# Autodesk Inventor assembly: Ensamblaje
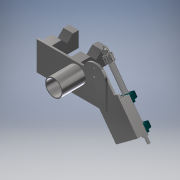
[picture p0: Inventor's stored thumbnail of the model, 180x180]
Saved by Autodesk Inventor 2018 (Build 220112000, 112)
## iProperties
Created: 2021-07-05
Part Number: Ensamblaje
Material: Genérico
Document SubType Name: Assembly
Designer: GABRIEL
Author: GABRIEL
## Documents named in this file (9)
- C:\Users\GABRIEL\Documents\Gabriel\UNAL\SEMESTRE XI\Automatización de PM\Proyecto\Maquina de boca de pescado\Ensamblaje.iam
- C:\Users\GABRIEL\Documents\Gabriel\Modelados\Placa1.ipt
- C:\Users\GABRIEL\Documents\Gabriel\UNAL\SEMESTRE XI\Automatización de PM\Proyecto\Maquina de boca de pescado\Base.ipt
- C:\Users\GABRIEL\Documents\Gabriel\UNAL\SEMESTRE XI\Automatización de PM\Proyecto\Maquina de boca de pescado\Posicionador.ipt
- C:\Users\GABRIEL\Documents\Gabriel\UNAL\SEMESTRE XI\Automatización de PM\Proyecto\Maquina de boca de pescado\pie.ipt
- C:\Users\GABRIEL\Documents\Gabriel\UNAL\SEMESTRE XI\Automatización de PM\Proyecto\Maquina de boca de pescado\24200-25205.iam
- C:\Users\GABRIEL\Documents\Gabriel\UNAL\SEMESTRE XI\Automatización de PM\Proyecto\Maquina de boca de pescado\Soporte_rods.ipt
- C:\Users\GABRIEL\Documents\Gabriel\UNAL\SEMESTRE XI\Automatización de PM\Proyecto\Maquina de boca de pescado\eje.ipt
- C:\Users\GABRIEL\Documents\Gabriel\UNAL\SEMESTRE XI\Automatización de PM\Proyecto\Maquina de boca de pescado\spindle.ipt
## Components (10 placed, 8 different names)
1. Base:1 — Coincidencia:1, Nivelación:1, Nivelación:2, Coincidencia:2, Nivelación:3, Coincidencia:6, Nivelación:4, Nivelación:5, Coincidencia:11, Coincidencia:12, Ángulo:1
2. Soporte:1 — Coincidencia:1, Nivelación:1, Nivelación:2, Coincidencia:3
3. Soporte:2 — Coincidencia:2, Nivelación:3, Coincidencia:3, Coincidencia:7
4. pie:1 — Coincidencia:6, Nivelación:4, Nivelación:5, Coincidencia:7
5. Posicionador:1 — Coincidencia:8, Nivelación:6, Nivelación:7, Coincidencia:11, Coincidencia:12, Ángulo:1
6. Rodamiento:1 [sub-assembly] — Coincidencia:9, Nivelación:8, Nivelación:9, Insertar:1
7. Rodamiento:2 [sub-assembly] — Coincidencia:10, Nivelación:10, Nivelación:11
8. Soporte_rods:1 — Coincidencia:8, Nivelación:6, Nivelación:7, Coincidencia:9, Nivelación:8, Nivelación:9, Coincidencia:10, Nivelación:10, Nivelación:11
9. eje:1 — Insertar:1, Coincidencia:13, Coincidencia:14, Rotación:1
10. spindle:1 — Coincidencia:13, Coincidencia:14, Rotación:1
## Relationships (26: Mate 12, Flush 11, Angle 1, Insert 1, RelateRotation 1)
- Coincidencia:1 [Mate]: Base:1 ↔ Soporte:1
- Nivelación:1 [Flush] (10 mm): Base:1 ↔ Soporte:1
- Nivelación:2 [Flush] (-10 mm): Base:1 ↔ Soporte:1
- Coincidencia:2 [Mate]: Base:1 ↔ Soporte:2
- Nivelación:3 [Flush] (10 mm): Base:1 ↔ Soporte:2
- Coincidencia:3 [Mate] (100 mm): Soporte:1 ↔ Soporte:2
- Coincidencia:6 [Mate]: Base:1 ↔ pie:1
- Nivelación:4 [Flush]: Base:1 ↔ pie:1
- Nivelación:5 [Flush] (10 mm): Base:1 ↔ pie:1
- Coincidencia:7 [Mate]: Soporte:2 ↔ pie:1
- Coincidencia:8 [Mate]: Posicionador:1 ↔ Soporte_rods:1
- Nivelación:6 [Flush]: Posicionador:1 ↔ Soporte_rods:1
- Nivelación:7 [Flush]: Posicionador:1 ↔ Soporte_rods:1
- Coincidencia:9 [Mate]: Rodamiento:1 ↔ Soporte_rods:1
- Nivelación:8 [Flush]: Rodamiento:1 ↔ Soporte_rods:1
- Nivelación:9 [Flush]: Rodamiento:1 ↔ Soporte_rods:1
- Coincidencia:10 [Mate]: Rodamiento:2 ↔ Soporte_rods:1
- Nivelación:10 [Flush]: Rodamiento:2 ↔ Soporte_rods:1
- Nivelación:11 [Flush]: Rodamiento:2 ↔ Soporte_rods:1
- Coincidencia:11 [Mate]: Base:1 ↔ Posicionador:1
- Coincidencia:12 [Mate]: Base:1 ↔ Posicionador:1
- Ángulo:1 [Angle] (0 deg): Base:1 ↔ Posicionador:1
- Insertar:1 (-20 mm): Rodamiento:1 ↔ eje:1
- Coincidencia:13 [Mate]: eje:1 ↔ spindle:1
- Coincidencia:14 [Mate]: eje:1 ↔ spindle:1
- Rotación:1 [RelateRotation] (1 ul): eje:1 ↔ spindle:1
